# Autodesk Inventor assembly: Assembly1
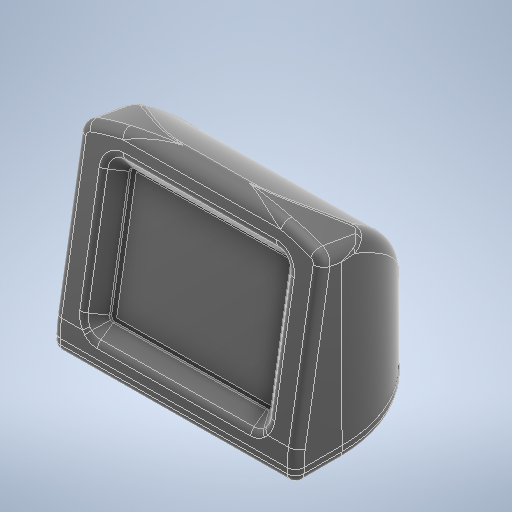
[picture p0: Inventor's stored thumbnail of the model, 512x512]
Saved by Autodesk Inventor 2025 (Build 290162000, 162)
## iProperties
Created: 2024-12-23
Part Number: Assembly1
Document SubType Name: Assembly
Designer: tvoko
Author: tvoko
## Documents named in this file (8)
- C:\Users\tvoko\Documents\GitHub\EternalEscape\Hardware\EternalEscapeMainAssy.iam
- C:\Users\tvoko\Documents\GitHub\EternalEscape\Hardware\Buyouts\2090 2.8in TFT Cap Touch.ipt
- C:\Users\tvoko\Documents\School\Fall 2024\Senior Design Pt 1\Lab 1\Buyouts\5323 Feather ESP32-S3\5323 Feather ESP32-S3.ipt
- C:\Users\tvoko\Documents\GitHub\EternalEscape\Hardware\Top.ipt
- C:\Users\tvoko\Documents\Inventor\Content Center Files\R2025\en-US\ISO 4762(2)\ISO 4762 - M3 x 5ISO.ipt
- C:\Users\tvoko\Documents\GitHub\EternalEscape\Hardware\Bottom.ipt
- C:\Users\tvoko\Documents\Inventor\Content Center Files\R2025\en-US\ISO 4762(2)\ISO 4762 - M3 x 8ISO.ipt
- C:\Users\tvoko\Documents\Inventor\Content Center Files\R2025\en-US\ISO 4762(2)\ISO 4762 - M2 x 3ISO.ipt
## Components (14 placed, 7 different names)
1. 2090 2.8in TFT Cap Touch:1 — Mate:1, Mate:2, Mate:5, Mate:6, Mate:7
2. 5323 Feather ESP32-S3:1 — Mate:9, Mate:10, Mate:15, Mate:17, Mate:18, Mate:19, Mate:20
3. Top:1 — Mate:1, Mate:2, Mate:3, Mate:4, Mate:7, Mate:8, Mate:21, Mate:22, Mate:23, Mate:24
4. ISO 4762 M3 x 5:1 — Mate:3, Mate:5
5. ISO 4762 M3 x 5:2 — Mate:4, Mate:6
6. Bottom:1 — Mate:8, Mate:9, Mate:10, Mate:11, Mate:12, Mate:13, Mate:14, Mate:15, Mate:16, Mate:21, Mate:22, Mate:23, Mate:24, Mate:25, Mate:26, Mate:27, Mate:28, Mate:29, Mate:30, Mate:31, Mate:32
7. ISO 4762 M2 x 3:1 — Mate:11, Mate:12, Mate:19
8. ISO 4762 M3 x 8:1 — Mate:27, Mate:32
9. ISO 4762 M3 x 8:2 — Mate:26, Mate:31
10. ISO 4762 M3 x 8:3 — Mate:28, Mate:29
11. ISO 4762 M3 x 8:4 — Mate:25, Mate:30
12. ISO 4762 M2 x 3:2 — Mate:13, Mate:20
13. ISO 4762 M2 x 3:3 — Mate:16, Mate:17
14. ISO 4762 M2 x 3:4 — Mate:14, Mate:18
## Relationships (32: Mate 32)
- Mate:1: 2090 2.8in TFT Cap Touch:1 ↔ Top:1
- Mate:2: 2090 2.8in TFT Cap Touch:1 ↔ Top:1
- Mate:3: Top:1 ↔ ISO 4762 M3 x 5:1
- Mate:4: Top:1 ↔ ISO 4762 M3 x 5:2
- Mate:5: 2090 2.8in TFT Cap Touch:1 ↔ ISO 4762 M3 x 5:1
- Mate:6: 2090 2.8in TFT Cap Touch:1 ↔ ISO 4762 M3 x 5:2
- Mate:7: 2090 2.8in TFT Cap Touch:1 ↔ Top:1
- Mate:8: Top:1 ↔ Bottom:1
- Mate:9: 5323 Feather ESP32-S3:1 ↔ Bottom:1
- Mate:10: 5323 Feather ESP32-S3:1 ↔ Bottom:1
- Mate:11: Bottom:1 ↔ ISO 4762 M2 x 3:1
- Mate:12: Bottom:1 ↔ ISO 4762 M2 x 3:1
- Mate:13: Bottom:1 ↔ ISO 4762 M2 x 3:2
- Mate:14: Bottom:1 ↔ ISO 4762 M2 x 3:4
- Mate:15: 5323 Feather ESP32-S3:1 ↔ Bottom:1
- Mate:16: Bottom:1 ↔ ISO 4762 M2 x 3:3
- Mate:17: 5323 Feather ESP32-S3:1 ↔ ISO 4762 M2 x 3:3
- Mate:18: 5323 Feather ESP32-S3:1 ↔ ISO 4762 M2 x 3:4
- Mate:19: 5323 Feather ESP32-S3:1 ↔ ISO 4762 M2 x 3:1
- Mate:20: 5323 Feather ESP32-S3:1 ↔ ISO 4762 M2 x 3:2
- Mate:21: Top:1 ↔ Bottom:1
- Mate:22: Top:1 ↔ Bottom:1
- Mate:23: Top:1 ↔ Bottom:1
- Mate:24: Top:1 ↔ Bottom:1
- Mate:25: Bottom:1 ↔ ISO 4762 M3 x 8:4
- Mate:26: Bottom:1 ↔ ISO 4762 M3 x 8:2
- Mate:27: Bottom:1 ↔ ISO 4762 M3 x 8:1
- Mate:28: Bottom:1 ↔ ISO 4762 M3 x 8:3
- Mate:29: Bottom:1 ↔ ISO 4762 M3 x 8:3
- Mate:30: Bottom:1 ↔ ISO 4762 M3 x 8:4
- Mate:31: Bottom:1 ↔ ISO 4762 M3 x 8:2
- Mate:32: Bottom:1 ↔ ISO 4762 M3 x 8:1
